# Autodesk Inventor assembly: cat
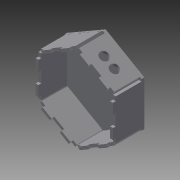
[picture p0: Inventor's stored thumbnail of the model, 180x180]
Saved by Autodesk Inventor 2015 (Build 190159000, 159)
## iProperties
Created: 2017-11-28
Part Number: cat
Document SubType Name: Assembly
Designer: Max
Author: Max
## Documents named in this file (4)
- C:\Users\Max\Dropbox\cat\cat.iam
- C:\Users\Max\Dropbox\cat\base.ipt
- C:\Users\Max\Dropbox\cat\cara.ipt
- C:\Users\Max\Dropbox\cat\lado.ipt
## Components (7 placed, 3 different names)
1. base:1 — Flush:1, Mate:1, Mate:2, Flush:2, Mate:3, Mate:4, Flush:3, Mate:5, Mate:6, Flush:4, Mate:7, Mate:8, Flush:5, Mate:9, Mate:10, Flush:6, Mate:11, Mate:12
2. cara:1 — Flush:1, Mate:1, Mate:2
3. lado:1 — Flush:3, Mate:5, Mate:6
4. lado:3 — Flush:4, Mate:7, Mate:8
5. lado:5 — Flush:2, Mate:3, Mate:4
6. lado:6 — Flush:5, Mate:9, Mate:10
7. lado:7 — Flush:6, Mate:11, Mate:12
## Relationships (18: Mate 12, Flush 6)
- Flush:1: base:1 ↔ cara:1
- Mate:1: base:1 ↔ cara:1
- Mate:2: base:1 ↔ cara:1
- Flush:2: base:1 ↔ lado:5
- Mate:3: base:1 ↔ lado:5
- Mate:4: base:1 ↔ lado:5
- Flush:3: base:1 ↔ lado:1
- Mate:5: base:1 ↔ lado:1
- Mate:6: base:1 ↔ lado:1
- Flush:4: base:1 ↔ lado:3
- Mate:7: base:1 ↔ lado:3
- Mate:8: base:1 ↔ lado:3
- Flush:5: base:1 ↔ lado:6
- Mate:9: base:1 ↔ lado:6
- Mate:10: base:1 ↔ lado:6
- Flush:6: base:1 ↔ lado:7
- Mate:11: base:1 ↔ lado:7
- Mate:12: base:1 ↔ lado:7
